# Autodesk Inventor assembly: KiCad-OBC
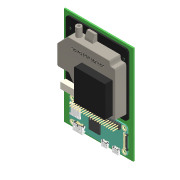
[picture p0: Inventor's stored thumbnail of the model, 180x180]
Saved by Autodesk Inventor 2022 (Build 260153000, 153)
## iProperties
Company: Kicad
Created: 2022-02-26
Part Number: KiCad-OBC
Description: KiCad electronic assembly
Document SubType Name: Assembly
Designer: admin
Authority: Unknown
Title: KiCad-OBC.step
Author: Pcbnew
Sending System: KiCad to STEP converter
Preprocessor: Open CASCADE STEP processor 7.6
## Documents named in this file (6)
- C:\Users\admin\Desktop\KiCad-OBC\Exports\KiCad-OBC.iam
- C:\Users\admin\Desktop\KiCad-OBC\Exports\HCLGA-10L_2P5X2P5X1_STM.iam
- C:\Users\admin\Desktop\KiCad-OBC\Exports\HLGA-6L_2X2_STM.iam
- C:\Users\admin\Desktop\KiCad-OBC\Exports\PMsensor_Nova_SDS011.iam
- C:\Users\admin\Desktop\KiCad-OBC\Exports\KiCad-OBC PCB.ipt
- C:\Users\admin\Desktop\KiCad-OBC\Parts\RPi Zero'\ADA3708.ipt
## Components (5 placed, 5 different names)
1. 2 [sub-assembly]
2. 4 [sub-assembly]
3. 6 [sub-assembly]
4. 7 — Mate:1, Mate:2
5. ADA3708:1 — Mate:1, Mate:2
## Relationships (2: Mate 2)
- Mate:1: 7 ↔ ADA3708:1
- Mate:2: 7 ↔ ADA3708:1
